# Autodesk Inventor assembly: NTBG6-4
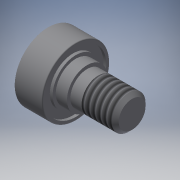
[picture p0: Inventor's stored thumbnail of the model, 180x180]
Saved by Autodesk Inventor 2019 (Build 230136000, 136)
## iProperties
Category: PARTsolutions
Company: MISUMI
Created: 2023-12-09
Part Number: NTBG6-4
Catalog Web Link: www.cadenas.de
Description: NTBG, NTSBG-Bearings with Male Threads
Vendor: MISUMI
Document SubType Name: Assembly
Designer: psAdmin
Manufacturer: MISUMI
Mass: 0.0999469 g
Surface Area: 2.23567 cm^2
Volume: 0.0999469 cm^3
Density: 1 g/cm^3
Title: NTBG6-4
Author: Cadenas PARTsolutions
Comments: Bearings with Male Threads
PSOL_IDENT_0: {$CADENAS_DATA/23d-libs/misumi/metric/53_rollers/ntsbg_asmtab.prj},168 {VTYP=3D},{STYP=ASSTAB},{NB=N
PSOL_IDENT_1: TBG6-4},{LINA=NTBG6-4},{NN=NTBG, NTSBG},{DATE=16.02.2023 07:07:41},{GEOMDATE=16.10.2013},{VERSION=},
PSOL_IDENT_2: {LINEID=10},{WBVAR=MATB},{WBNUMERIC=}  {NB=NTBG6-4},{LINA=NTBG6-4},{KT=DUMMY},{PN=NTBG6-4},{TYPE=NTB
PSOL_IDENT_3: G},{TS=},{MATB=},{MATB1= '', 'Steel', 'S', 'Stainless Steel' },{MATS=SUM},{ST=Electroless Nickel Pla
PSOL_IDENT_4: ting},{D=6},{L=4},{B=2.5},{DD=3},{AA=1.0},{G=1.5},{M=M3},{M1=3},{BE=673ZZ},{LSM=4},{LLM=0},{D1=3.600
PSOL_IDENT_5: },{B1=2.4200},{G1=1.5},{DIA=0.080},{PPATH=ntbg_asmtpl.prj},{Z=0.2}
NB: NTBG6-4
NN: NTBG, NTSBG
NT: Bearings with Male Threads
NBSYN: $PN.
LINA: NTBG6-4
CATALOG: Misumi
PN: NTBG6-4
MATB: Steel
ST: Electroless Nickel Plating
D: 6
L: 4
B: 2.5
DD: 3
AA: 1
G: 1.5
M: M3
BE: 673ZZ
SUPPLIER: MISUMI
ARTICLENO: NTBG6-4
BOMINFO: NTBG6-4
CREATOR: CADENAS GmbH
## Documents named in this file (3)
- e:\temp\worker_COMMON_2\temp\tmp_8124_18_2wk81\format_0\NTBG6-4.iam
- e:\temp\worker_COMMON_2\temp\tmp_8124_18_2wk81\format_0\NTBG6-4_a.ipt
- e:\temp\worker_COMMON_2\temp\tmp_8124_18_2wk81\format_0\B673ZZ.ipt
## Components (2 placed, 2 different names)
1. NTBG6-4_a:1 — shaft_to_bearing_XY@1 <-> to_housing_XY@2, shaft_to_bearing_Z@1 <-> to_housing_Z@2, shaft_to_bearing_YZ@1 <-> to_housing_YZ@2
2. B673ZZ:1 — shaft_to_bearing_XY@1 <-> to_housing_XY@2, shaft_to_bearing_Z@1 <-> to_housing_Z@2, shaft_to_bearing_YZ@1 <-> to_housing_YZ@2
## Relationships (3: Mate 2, Angle 1)
- shaft_to_bearing_XY@1 <-> to_housing_XY@2 [Mate]: NTBG6-4_a:1 ↔ B673ZZ:1
- shaft_to_bearing_Z@1 <-> to_housing_Z@2 [Mate]: NTBG6-4_a:1 ↔ B673ZZ:1
- shaft_to_bearing_YZ@1 <-> to_housing_YZ@2 [Angle] (0 deg): NTBG6-4_a:1 ↔ B673ZZ:1
